# Autodesk Inventor assembly: Assieme
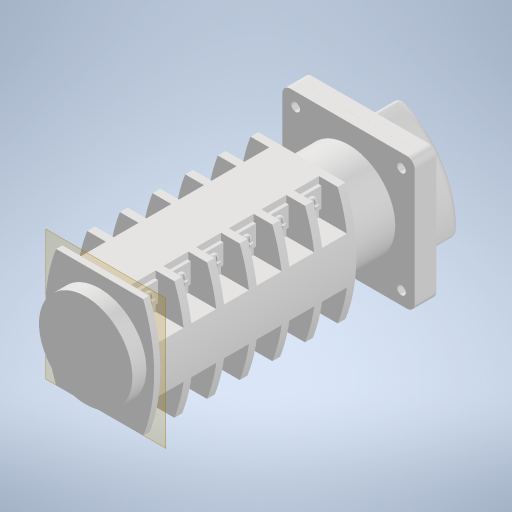
[picture p0: Inventor's stored thumbnail of the model, 512x512]
Saved by Autodesk Inventor 2024 (Build 280153000, 153)
## iProperties
Created: 2023-12-19
Part Number: Assieme
Document SubType Name: Assembly
Designer: cecca
Author: cecca
## Documents named in this file (7)
- C:\Users\cecca\OneDrive - Università Politecnica delle Marche\UNIVPM\Erasmus\2 Design\Progetto\Assieme.iam
- C:\Users\cecca\OneDrive - Università Politecnica delle Marche\UNIVPM\Erasmus\2 Design\Progetto\Parte1.ipt
- C:\Users\cecca\OneDrive - Università Politecnica delle Marche\UNIVPM\Erasmus\2 Design\Progetto\Parte2.ipt
- C:\Users\cecca\OneDrive - Università Politecnica delle Marche\UNIVPM\Erasmus\2 Design\Progetto\Parte3.ipt
- C:\Users\cecca\OneDrive - Università Politecnica delle Marche\UNIVPM\Erasmus\2 Design\Progetto\Parte4.ipt
- C:\Users\cecca\OneDrive - Università Politecnica delle Marche\UNIVPM\Erasmus\2 Design\Progetto\Parte5.ipt
- C:\Users\cecca\OneDrive - Università Politecnica delle Marche\UNIVPM\Erasmus\2 Design\Progetto\Parte6.ipt
## Components (6 placed, 6 different names)
1. Parte1:1 — Coincidente:1, Coincidente:2, Coincidente:3, Rotazionale:1, Rotazionale:2
2. Parte2:1 — Coincidente:3
3. Parte3:1 — Rotazionale:1, Rotazionale:3
4. Parte4:1 — Rotazionale:2
5. Parte5:1 — Rotazionale:3
6. Parte6:1 — Coincidente:1, Coincidente:2
## Relationships (6: Mate 3, RevoluteJoint 3)
- Coincidente:1 [Mate]: Parte1:1 ↔ Parte6:1
- Coincidente:2 [Mate]: Parte1:1 ↔ Parte6:1
- Coincidente:3 [Mate]: Parte1:1 ↔ Parte2:1
- Rotazionale:1 [RevoluteJoint]: Parte1:1 ↔ Parte3:1
- Rotazionale:2 [RevoluteJoint]: Parte1:1 ↔ Parte4:1
- Rotazionale:3 [RevoluteJoint]: Parte3:1 ↔ Parte5:1
